# Autodesk Inventor assembly: ResGalvoScanAssembly
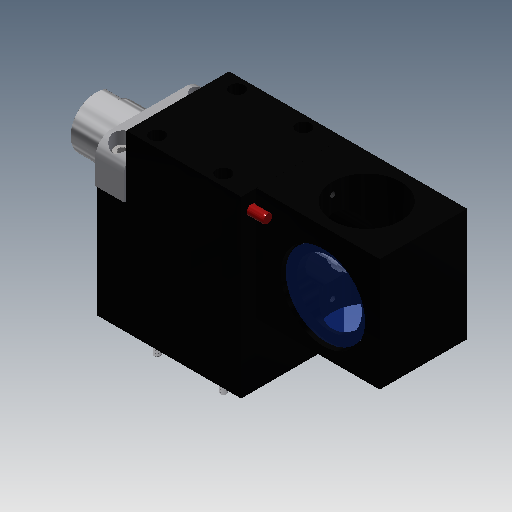
[picture p0: Inventor's stored thumbnail of the model, 512x512]
Saved by Autodesk Inventor 2018.2 (Build 222227000, 227)
## iProperties
Created: 2018-06-06
Part Number: ResGalvoScanAssembly
Document SubType Name: Assembly
Designer: legant_local
Author: legant_local
## Documents named in this file (11)
- E:\AOLLS_SVN\workspace\Sub assemblies\ResGalvoScanAssembly.iam
- E:\AOLLS_SVN\workspace\Imported Components\McMaster_Carr\McMaster_Carr_91585A351_dowel_pin_D3mm_L10mm.ipt
- E:\AOLLS_SVN\workspace\Imported Components\Thorlabs\Thorlabs_20-1531-001_ResGalvoClamp.ipt
- E:\AOLLS_SVN\workspace\Imported Components\Edmund\Edmund_36997_D25mm_T1mm_VISNIR_Window.ipt
- E:\AOLLS_SVN\workspace\Imported Components\McMaster_Carr\McMaster_Carr_92290A747_M2x20mm_socket_cap.ipt
- E:\AOLLS_SVN\workspace\Imported Components\McMaster_Carr\McMaster_Carr_92290A115_M3x10mm_socket_cap.ipt
- E:\AOLLS_SVN\workspace\Imported Components\Misumi\Misumi steel diamond pin JPDB3-4.ipt
- E:\AOLLS_SVN\workspace\Imported Components\Misumi\Misumi steel round      pin JPBB3-4.ipt
- E:\AOLLS_SVN\workspace\Imported Components\Cambridge_Technology\CRS08K-S3-S-045 CRS 8kHz.ipt
- E:\AOLLS_SVN\workspace\Custom Parts Linked With Drawings\Main Assembly\ResGalvoWindow.ipt
- E:\AOLLS_SVN\workspace\Custom Parts Linked With Drawings\Main Assembly\ResGalvoMount_scan.ipt
## Components (19 placed, 10 different names)
1. CRS08K-S3-S-045 CRS 8kHz:1 — Mate:31, Angle:3, Mate:32, Angle:4, Mate:33
2. ResGalvoMount_scan:1 — Mate:2, Flush:2, Flush:3, Mate:3, Mate:4, Flush:4, Flush:5, Mate:5, Flush:6, Mate:7, Mate:8, Flush:7, Mate:13, Mate:14, Mate:15, Mate:16, Mate:17, Mate:18, Mate:19, Mate:20, Mate:21, Mate:22, Mate:23, Mate:24, Mate:29, Mate:30, Flush:8, Flush:9, Angle:2, Mate:31, Angle:3, Mate:32, Angle:4, Mate:33
3. ResGalvoWindow:1 — Mate:2, Flush:2, Flush:3, Mate:9, Mate:10, Mate:11, Mate:12
4. Misumi steel diamond pin JPDB3-4:1 — Mate:29, Flush:8, Angle:2
5. Misumi steel round      pin JPBB3-4:1 — Mate:30, Flush:9
6. McMaster_Carr_91585A351_dowel_pin_D3mm_L10mm:1 — Mate:4, Flush:4
7. McMaster_Carr_91585A351_dowel_pin_D3mm_L10mm:2 — Mate:3, Flush:5
8. McMaster_Carr_91585A351_dowel_pin_D3mm_L10mm:3 — Mate:5, Flush:6
9. Thorlabs_20-1531-001_ResGalvoClamp:1 — Mate:7, Mate:8, Flush:7, Mate:25, Mate:26, Mate:27, Mate:28
10. Edmund_36997_D25mm_T1mm_VISNIR_Window:1 — Mate:9, Mate:10
11. Edmund_36997_D25mm_T1mm_VISNIR_Window:2 — Mate:11, Mate:12
12. McMaster_Carr_92290A747_M2x20mm_socket_cap:1 — Mate:13, Mate:14
13. McMaster_Carr_92290A747_M2x20mm_socket_cap:2 — Mate:15, Mate:20
14. McMaster_Carr_92290A747_M2x20mm_socket_cap:3 — Mate:16, Mate:19
15. McMaster_Carr_92290A747_M2x20mm_socket_cap:4 — Mate:17, Mate:18
16. McMaster_Carr_92290A747_M2x20mm_socket_cap:5 — Mate:21, Mate:24
17. McMaster_Carr_92290A747_M2x20mm_socket_cap:6 — Mate:22, Mate:23
18. McMaster_Carr_92290A115_M3x10mm_socket_cap:1 — Mate:25, Mate:26
19. McMaster_Carr_92290A115_M3x10mm_socket_cap:2 — Mate:27, Mate:28
## Relationships (42: Mate 31, Flush 8, Angle 3)
- Mate:2: ResGalvoMount_scan:1 ↔ ResGalvoWindow:1
- Flush:2: ResGalvoMount_scan:1 ↔ ResGalvoWindow:1
- Flush:3: ResGalvoMount_scan:1 ↔ ResGalvoWindow:1
- Mate:3: ResGalvoMount_scan:1 ↔ McMaster_Carr_91585A351_dowel_pin_D3mm_L10mm:2
- Mate:4: ResGalvoMount_scan:1 ↔ McMaster_Carr_91585A351_dowel_pin_D3mm_L10mm:1
- Flush:4 (-5 mm): ResGalvoMount_scan:1 ↔ McMaster_Carr_91585A351_dowel_pin_D3mm_L10mm:1
- Flush:5 (-5 mm): ResGalvoMount_scan:1 ↔ McMaster_Carr_91585A351_dowel_pin_D3mm_L10mm:2
- Mate:5: ResGalvoMount_scan:1 ↔ McMaster_Carr_91585A351_dowel_pin_D3mm_L10mm:3
- Flush:6 (-5 mm): ResGalvoMount_scan:1 ↔ McMaster_Carr_91585A351_dowel_pin_D3mm_L10mm:3
- Mate:7: ResGalvoMount_scan:1 ↔ Thorlabs_20-1531-001_ResGalvoClamp:1
- Mate:8: ResGalvoMount_scan:1 ↔ Thorlabs_20-1531-001_ResGalvoClamp:1
- Flush:7: ResGalvoMount_scan:1 ↔ Thorlabs_20-1531-001_ResGalvoClamp:1
- Mate:9: ResGalvoWindow:1 ↔ Edmund_36997_D25mm_T1mm_VISNIR_Window:1
- Mate:10: ResGalvoWindow:1 ↔ Edmund_36997_D25mm_T1mm_VISNIR_Window:1
- Mate:11: ResGalvoWindow:1 ↔ Edmund_36997_D25mm_T1mm_VISNIR_Window:2
- Mate:12: ResGalvoWindow:1 ↔ Edmund_36997_D25mm_T1mm_VISNIR_Window:2
- Mate:13: ResGalvoMount_scan:1 ↔ McMaster_Carr_92290A747_M2x20mm_socket_cap:1
- Mate:14: ResGalvoMount_scan:1 ↔ McMaster_Carr_92290A747_M2x20mm_socket_cap:1
- Mate:15: ResGalvoMount_scan:1 ↔ McMaster_Carr_92290A747_M2x20mm_socket_cap:2
- Mate:16: ResGalvoMount_scan:1 ↔ McMaster_Carr_92290A747_M2x20mm_socket_cap:3
- Mate:17: ResGalvoMount_scan:1 ↔ McMaster_Carr_92290A747_M2x20mm_socket_cap:4
- Mate:18: ResGalvoMount_scan:1 ↔ McMaster_Carr_92290A747_M2x20mm_socket_cap:4
- Mate:19: ResGalvoMount_scan:1 ↔ McMaster_Carr_92290A747_M2x20mm_socket_cap:3
- Mate:20: ResGalvoMount_scan:1 ↔ McMaster_Carr_92290A747_M2x20mm_socket_cap:2
- Mate:21: ResGalvoMount_scan:1 ↔ McMaster_Carr_92290A747_M2x20mm_socket_cap:5
- Mate:22: ResGalvoMount_scan:1 ↔ McMaster_Carr_92290A747_M2x20mm_socket_cap:6
- Mate:23: ResGalvoMount_scan:1 ↔ McMaster_Carr_92290A747_M2x20mm_socket_cap:6
- Mate:24: ResGalvoMount_scan:1 ↔ McMaster_Carr_92290A747_M2x20mm_socket_cap:5
- Mate:25: Thorlabs_20-1531-001_ResGalvoClamp:1 ↔ McMaster_Carr_92290A115_M3x10mm_socket_cap:1
- Mate:26: Thorlabs_20-1531-001_ResGalvoClamp:1 ↔ McMaster_Carr_92290A115_M3x10mm_socket_cap:1
- Mate:27: Thorlabs_20-1531-001_ResGalvoClamp:1 ↔ McMaster_Carr_92290A115_M3x10mm_socket_cap:2
- Mate:28: Thorlabs_20-1531-001_ResGalvoClamp:1 ↔ McMaster_Carr_92290A115_M3x10mm_socket_cap:2
- Mate:29: ResGalvoMount_scan:1 ↔ Misumi steel diamond pin JPDB3-4:1
- Mate:30: ResGalvoMount_scan:1 ↔ Misumi steel round      pin JPBB3-4:1
- Flush:8: ResGalvoMount_scan:1 ↔ Misumi steel diamond pin JPDB3-4:1
- Flush:9: ResGalvoMount_scan:1 ↔ Misumi steel round      pin JPBB3-4:1
- Angle:2 (0 deg): ResGalvoMount_scan:1 ↔ Misumi steel diamond pin JPDB3-4:1
- Mate:31 (-35 mm): CRS08K-S3-S-045 CRS 8kHz:1 ↔ ResGalvoMount_scan:1
- Angle:3 (0 deg): CRS08K-S3-S-045 CRS 8kHz:1 ↔ ResGalvoMount_scan:1
- Mate:32 (20.559 mm): CRS08K-S3-S-045 CRS 8kHz:1 ↔ ResGalvoMount_scan:1
- Angle:4 (-45 deg): CRS08K-S3-S-045 CRS 8kHz:1 ↔ ResGalvoMount_scan:1
- Mate:33: CRS08K-S3-S-045 CRS 8kHz:1 ↔ ResGalvoMount_scan:1
